# Autodesk Inventor assembly: MechanicalHand
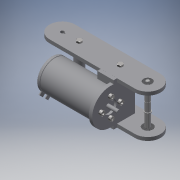
[picture p0: Inventor's stored thumbnail of the model, 180x180]
Saved by Autodesk Inventor 2018 (Build 220112000, 112)
## iProperties
Created: 2017-05-31
Part Number: MechanicalHand
Document SubType Name: Weldment
Designer: Damian
Weld Material: Welded Aluminum-6061
Author: Damian
## Documents named in this file (10)
- C:\Users\Damian\MechanicalHand\CAD\MechanicalFinger.iam
- C:\Users\Damian\MechanicalHand\StandardParts\3564_B\3564_B.ipt
- C:\Users\Damian\MechanicalHand\CAD\BaseJointMotorMount.ipt
- C:\Users\Damian\MechanicalHand\CAD\BaseJointPlate.ipt
- C:\Users\Damian\MechanicalHand\CAD\BushingSmall.ipt
- C:\Users\Damian\MechanicalHand\CAD\BushingLarge.ipt
- C:\Users\Damian\MechanicalHand\StandardParts\Bearing\Bearing.ipt
- C:\Users\Damian\MechanicalHand\CAD\ShortShaft\JointShaft.ipt
- C:\Users\Damian\Documents\Inventor\Content Center Files\R2018\en-US\AS 1110\AS 1110 - M3 x 6.ipt
- C:\Users\Damian\Documents\Inventor\Content Center Files\R2018\en-US\AS 1420\AS 1420 - 1973 - M3 x 6.ipt
## Components (17 placed, 9 different names)
1. 3564_B:1 — Mate:1, Mate:2, Mate:3
2. BaseJointMotorMount:1 — Mate:1, Mate:2, Mate:3, Mate:4, Mate:5, Mate:6, Mate:7, Mate:9, Mate:17, Insert:5, Mate:24
3. BaseJointPlate:1 — Mate:4, Mate:5, Mate:11, Mate:14, Mate:16, Mate:17, Insert:3, Insert:4
4. BaseJointPlate:2 — Mate:6, Mate:7, Mate:8, Mate:10, Mate:12, Mate:13, Mate:15, Insert:1, Insert:2, Mate:22, Mate:23
5. BushingSmall:1 — Mate:8, Mate:9
6. BushingLarge:1 — Mate:10, Mate:11, Mate:12
7. Bearing:1 — Mate:13, Mate:15, Mate:18
8. Bearing:2 — Mate:14, Mate:16, Mate:19
9. JointShaft:1 — Mate:18, Mate:19
10. AS 1110 - Metric M3 x 6:1 — Insert:1
11. AS 1110 - Metric M3 x 6:2 — Insert:2
12. AS 1110 - Metric M3 x 6:3 — Insert:3
13. AS 1110 - Metric M3 x 6:4 — Insert:4
14. AS 1420 - Metric M3 x 6:1 — Insert:5
15. AS 1420 - Metric M3 x 6:2
16. AS 1420 - Metric M3 x 6:3
17. AS 1420 - Metric M3 x 6:4
## Component patterns: (4 elements, first: AS 1420 - Metric M3 x 6:1)
## Relationships (27: Mate 22, Insert 5)
- Mate:1: 3564_B:1 ↔ BaseJointMotorMount:1
- Mate:2: 3564_B:1 ↔ BaseJointMotorMount:1
- Mate:3: 3564_B:1 ↔ BaseJointMotorMount:1
- Mate:4: BaseJointMotorMount:1 ↔ BaseJointPlate:1
- Mate:5: BaseJointMotorMount:1 ↔ BaseJointPlate:1
- Mate:6: BaseJointMotorMount:1 ↔ BaseJointPlate:2
- Mate:7: BaseJointMotorMount:1 ↔ BaseJointPlate:2
- Mate:8: BaseJointPlate:2 ↔ BushingSmall:1
- Mate:9: BaseJointMotorMount:1 ↔ BushingSmall:1
- Mate:10: BaseJointPlate:2 ↔ BushingLarge:1
- Mate:11: BaseJointPlate:1 ↔ BushingLarge:1
- Mate:12: BaseJointPlate:2 ↔ BushingLarge:1
- Mate:13: BaseJointPlate:2 ↔ Bearing:1
- Mate:14: BaseJointPlate:1 ↔ Bearing:2
- Mate:15: BaseJointPlate:2 ↔ Bearing:1
- Mate:16: BaseJointPlate:1 ↔ Bearing:2
- Mate:17: BaseJointMotorMount:1 ↔ BaseJointPlate:1
- Mate:18: Bearing:1 ↔ JointShaft:1
- Mate:19: Bearing:2 ↔ JointShaft:1
- Insert:1: BaseJointPlate:2 ↔ AS 1110 - Metric M3 x 6:1
- Insert:2: BaseJointPlate:2 ↔ AS 1110 - Metric M3 x 6:2
- Insert:3: BaseJointPlate:1 ↔ AS 1110 - Metric M3 x 6:3
- Insert:4: BaseJointPlate:1 ↔ AS 1110 - Metric M3 x 6:4
- Insert:5: BaseJointMotorMount:1 ↔ AS 1420 - Metric M3 x 6:1
- Mate:22: BaseJointPlate:2
- Mate:23: BaseJointPlate:2
- Mate:24: BaseJointMotorMount:1
